# Autodesk Inventor assembly: Prototype Assembly
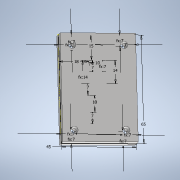
[picture p0: Inventor's stored thumbnail of the model, 180x180]
Saved by Autodesk Inventor 2021 (Build 250183000, 183)
## iProperties
Created: 2020-08-09
Part Number: Prototype Assembly
Document SubType Name: Assembly
Designer: natha
Author: natha
## Documents named in this file (3)
- C:\03_Dokumente\02_Master_Uni_Stuttgart\06_Studienarbeit Ausland\02_Work\04_CAD\Simple Prototype\Prototype Assembly.iam
- C:\03_Dokumente\02_Master_Uni_Stuttgart\06_Studienarbeit Ausland\02_Work\04_CAD\Simple Prototype\Prototype Flow Layer.ipt
- C:\03_Dokumente\02_Master_Uni_Stuttgart\06_Studienarbeit Ausland\02_Work\04_CAD\Simple Prototype\Prototype Control Layer1.ipt
## Components (2 placed, 2 different names)
1. Prototype Flow Layer:1 — Mate:1
2. Prototype Control Layer1:1 — Mate:1
## Relationships (1: Mate 1)
- Mate:1: Prototype Flow Layer:1 ↔ Prototype Control Layer1:1
